# Autodesk Inventor assembly: Power_PCB
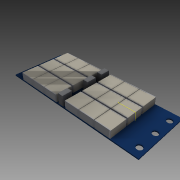
[picture p0: Inventor's stored thumbnail of the model, 180x180]
Saved by Autodesk Inventor 2016 (Build 200138000, 138)
## iProperties
Company: Open CASCADE
Created: 2015-06-05
Part Number: Power_PCB
Description: Open CASCADE Model
Document SubType Name: Assembly
Designer: Yann
Authority: Unknown
Title: Open CASCADE Shape Model
Author: Author
Sending System: Open CASCADE 6.5
Preprocessor: Open CASCADE STEP processor 6.5
## Documents named in this file (47)
- C:\Users\Yann\Documents\GitHub\BIKAIR_CAD\Source\Powertrain_Controller\Power_PCB.iam
- C:\Users\Yann\Documents\GitHub\BIKAIR_CAD\Source\Powertrain_Controller\Board.ipt
- C:\Users\Yann\Documents\GitHub\BIKAIR_CAD\Source\Powertrain_Controller\C1.iam
- C:\Users\Yann\Documents\GitHub\BIKAIR_CAD\Source\Powertrain_Controller\C2.iam
- C:\Users\Yann\Documents\GitHub\BIKAIR_CAD\Source\Powertrain_Controller\C3.iam
- C:\Users\Yann\Documents\GitHub\BIKAIR_CAD\Source\Powertrain_Controller\C4.iam
- C:\Users\Yann\Documents\GitHub\BIKAIR_CAD\Source\Powertrain_Controller\C5.iam
- C:\Users\Yann\Documents\GitHub\BIKAIR_CAD\Source\Powertrain_Controller\C6.iam
- C:\Users\Yann\Documents\GitHub\BIKAIR_CAD\Source\Powertrain_Controller\C7.iam
- C:\Users\Yann\Documents\GitHub\BIKAIR_CAD\Source\Powertrain_Controller\C8.iam
- C:\Users\Yann\Documents\GitHub\BIKAIR_CAD\Source\Powertrain_Controller\C9.iam
- C:\Users\Yann\Documents\GitHub\BIKAIR_CAD\Source\Powertrain_Controller\C10.iam
- C:\Users\Yann\Documents\GitHub\BIKAIR_CAD\Source\Powertrain_Controller\C11.iam
- C:\Users\Yann\Documents\GitHub\BIKAIR_CAD\Source\Powertrain_Controller\C12.iam
- C:\Users\Yann\Documents\GitHub\BIKAIR_CAD\Source\Powertrain_Controller\C13.iam
- C:\Users\Yann\Documents\GitHub\BIKAIR_CAD\Source\Powertrain_Controller\C14.iam
- C:\Users\Yann\Documents\GitHub\BIKAIR_CAD\Source\Powertrain_Controller\C15.iam
- C:\Users\Yann\Documents\GitHub\BIKAIR_CAD\Source\Powertrain_Controller\C16.iam
- C:\Users\Yann\Documents\GitHub\BIKAIR_CAD\Source\Powertrain_Controller\C17.iam
- C:\Users\Yann\Documents\GitHub\BIKAIR_CAD\Source\Powertrain_Controller\C18.iam
- C:\Users\Yann\Documents\GitHub\BIKAIR_CAD\Source\Powertrain_Controller\Q1.iam
- C:\Users\Yann\Documents\GitHub\BIKAIR_CAD\Source\Powertrain_Controller\Q2.iam
- C:\Users\Yann\Documents\GitHub\BIKAIR_CAD\Source\Powertrain_Controller\Q3.iam
- C:\Users\Yann\Documents\GitHub\BIKAIR_CAD\Source\Powertrain_Controller\Q4.iam
- C:\Users\Yann\Documents\GitHub\BIKAIR_CAD\Source\Powertrain_Controller\Q5.iam
- C:\Users\Yann\Documents\GitHub\BIKAIR_CAD\Source\Powertrain_Controller\Q6.iam
- C:\Users\Yann\Documents\GitHub\BIKAIR_CAD\Source\Powertrain_Controller\Q7.iam
- C:\Users\Yann\Documents\GitHub\BIKAIR_CAD\Source\Powertrain_Controller\Q8.iam
- C:\Users\Yann\Documents\GitHub\BIKAIR_CAD\Source\Powertrain_Controller\Q9.iam
- C:\Users\Yann\Documents\GitHub\BIKAIR_CAD\Source\Powertrain_Controller\Q10.iam
- C:\Users\Yann\Documents\GitHub\BIKAIR_CAD\Source\Powertrain_Controller\Q11.iam
- C:\Users\Yann\Documents\GitHub\BIKAIR_CAD\Source\Powertrain_Controller\Q12.iam
- C:\Users\Yann\Documents\GitHub\BIKAIR_CAD\Source\Powertrain_Controller\Q13.iam
- C:\Users\Yann\Documents\GitHub\BIKAIR_CAD\Source\Powertrain_Controller\Q14.iam
- C:\Users\Yann\Documents\GitHub\BIKAIR_CAD\Source\Powertrain_Controller\Q15.iam
- C:\Users\Yann\Documents\GitHub\BIKAIR_CAD\Source\Powertrain_Controller\Q16.iam
- C:\Users\Yann\Documents\GitHub\BIKAIR_CAD\Source\Powertrain_Controller\Q17.iam
- C:\Users\Yann\Documents\GitHub\BIKAIR_CAD\Source\Powertrain_Controller\Q18.iam
- C:\Users\Yann\Documents\GitHub\BIKAIR_CAD\Source\Powertrain_Controller\Q19.iam
- C:\Users\Yann\Documents\GitHub\BIKAIR_CAD\Source\Powertrain_Controller\Q20.iam
- C:\Users\Yann\Documents\GitHub\BIKAIR_CAD\Source\Powertrain_Controller\Q21.iam
- C:\Users\Yann\Documents\GitHub\BIKAIR_CAD\Source\Powertrain_Controller\Q22.iam
- C:\Users\Yann\Documents\GitHub\BIKAIR_CAD\Source\Powertrain_Controller\Q23.iam
- C:\Users\Yann\Documents\GitHub\BIKAIR_CAD\Source\Powertrain_Controller\Q24.iam
- C:\Users\Yann\Documents\GitHub\BIKAIR_CAD\Source\Powertrain_Controller\U_CONN.iam
- C:\Users\Yann\Documents\GitHub\BIKAIR_CAD\Source\Powertrain_Controller\V_CONN.iam
- C:\Users\Yann\Documents\GitHub\BIKAIR_CAD\Source\Powertrain_Controller\W_CONN.iam
## Components (46 placed, 46 different names)
1. 1
2. 7 [sub-assembly]
3. 11 [sub-assembly]
4. 15 [sub-assembly]
5. 19 [sub-assembly]
6. 23 [sub-assembly]
7. 27 [sub-assembly]
8. 31 [sub-assembly]
9. 35 [sub-assembly]
10. 39 [sub-assembly]
11. 43 [sub-assembly]
12. 47 [sub-assembly]
13. 51 [sub-assembly]
14. 55 [sub-assembly]
15. 59 [sub-assembly]
16. 63 [sub-assembly]
17. 67 [sub-assembly] — Symmetry:1
18. 71 [sub-assembly]
19. 75 [sub-assembly] — Symmetry:1
20. 80 [sub-assembly]
21. 83 [sub-assembly]
22. 86 [sub-assembly]
23. 89 [sub-assembly]
24. 94 [sub-assembly]
25. 98 [sub-assembly]
26. 101 [sub-assembly]
27. 104 [sub-assembly]
28. 108 [sub-assembly]
29. 111 [sub-assembly]
30. 114 [sub-assembly]
31. 117 [sub-assembly]
32. 120 [sub-assembly]
33. 123 [sub-assembly]
34. 126 [sub-assembly]
35. 129 [sub-assembly]
36. 132 [sub-assembly]
37. 135 [sub-assembly]
38. 138 [sub-assembly]
39. 141 [sub-assembly]
40. 144 [sub-assembly]
41. 147 [sub-assembly]
42. 150 [sub-assembly]
43. 153 [sub-assembly]
44. 156 [sub-assembly]
45. 158 [sub-assembly]
46. 160 [sub-assembly]
## Relationships (1: Symmetry 1)
- Symmetry:1: 67 ↔ 75
